# Autodesk Inventor assembly: feedCableStay
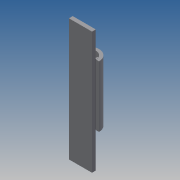
[picture p0: Inventor's stored thumbnail of the model, 180x180]
Saved by Autodesk Inventor 2014 SP1 (Build 180222100, 222)
## iProperties
Created: 2014-08-29
Part Number: feedCableStay
Document SubType Name: Assembly
Designer: Dave
Author: Dave
## Documents named in this file (3)
- C:\Users\Dave\Desktop\hera-cad\support\feedCableStay.iam
- C:\Users\Dave\Desktop\hera-cad\support\feedCableStay1.ipt
- C:\Users\Dave\Desktop\hera-cad\support\feedCableStay2.ipt
## Components (2 placed, 2 different names)
1. feedCableStay1:1 — Mate:1, Flush:1
2. feedCableStay2:1 — Mate:1, Flush:1
## Relationships (2: Mate 1, Flush 1)
- Mate:1 (-2.54 mm): feedCableStay1:1 ↔ feedCableStay2:1
- Flush:1: feedCableStay1:1 ↔ feedCableStay2:1
